# Autodesk Inventor assembly: Ring_1050_Sub
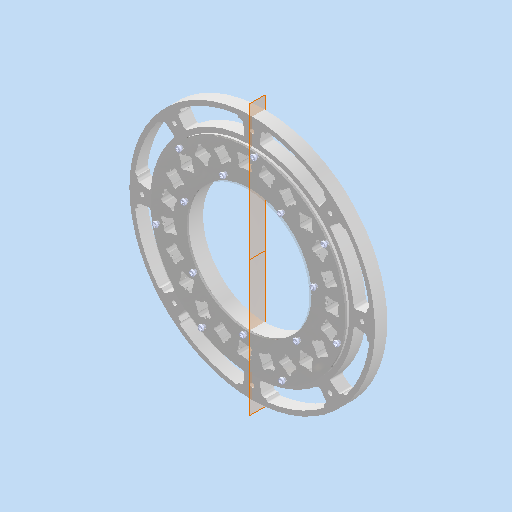
[picture p0: Inventor's stored thumbnail of the model, 512x512]
Saved by Autodesk Inventor 2024.2 (Build 282272000, 272)
## iProperties
Created: 2025-04-30
Part Number: Ring_1050_Sub
Document SubType Name: Assembly
Designer: 23661194
Author: 23661194
## Documents named in this file (4)
- C:\Users\23661194\OneDrive - Stellenbosch University\Master 2025 - Rat Scanner (120mm)\Rat_Scanner_120_V1\Ring_1050_Sub.iam
- C:\Users\23661194\OneDrive - Stellenbosch University\Master 2025 - Rat Scanner (120mm)\Rat_Scanner_120_V1\Ring_1050.ipt
- C:\Users\23661194\OneDrive - Stellenbosch University\Master 2025 - Rat Scanner (120mm)\Rat_Scanner_120_V1\Lid_Loose.ipt
- C:\Users\23661194\OneDrive - Stellenbosch University\Master 2025 - Rat Scanner (120mm)\Rat_Scanner_120_V1\M3x8.ipt
## Components (16 placed, 3 different names)
1. Ring_1050:1 — Mate:1, Mate:2, Mate:3, Mate:4, Mate:6
2. Lid_Loose:1 — Mate:1, Mate:2, Mate:3, Mate:5, Mate:7
3. M3x8:1 — Mate:4, Mate:5
4. M3x8:2
5. M3x8:3
6. M3x8:4
7. M3x8:5
8. M3x8:6
9. M3x8:7
10. M3x8:8 — Mate:6, Mate:7
11. M3x8:9
12. M3x8:10
13. M3x8:11
14. M3x8:12
15. M3x8:13
16. M3x8:14
## Component patterns: (7 elements, first: M3x8:1), (7 elements, first: M3x8:8)
## Relationships (7: Mate 7)
- Mate:1: Ring_1050:1 ↔ Lid_Loose:1
- Mate:2: Ring_1050:1 ↔ Lid_Loose:1
- Mate:3: Ring_1050:1 ↔ Lid_Loose:1
- Mate:4: Ring_1050:1 ↔ M3x8:1
- Mate:5: Lid_Loose:1 ↔ M3x8:1
- Mate:6: Ring_1050:1 ↔ M3x8:8
- Mate:7: Lid_Loose:1 ↔ M3x8:8
